# Autodesk Inventor assembly: Assembly2 (Intake Pipe Sub Assembly)
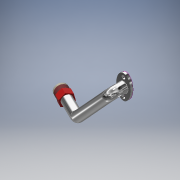
[picture p0: Inventor's stored thumbnail of the model, 180x180]
Saved by Autodesk Inventor 2018 (Build 220112000, 112)
## iProperties
Created: 2023-04-15
Part Number: Assembly2 (Intake Pipe Sub Assembly)
Document SubType Name: Assembly
Designer: Habib Mohamed
Author: Habib Mohamed
## Documents named in this file (5)
- D:\Inventor\My projects\Rotary Engine\Assembly\Assembly2 (Intake Pipe Sub Assembly).iam
- D:\Inventor\My projects\Rotary Engine\Component 51(Intake Pipe).ipt
- D:\Inventor\My projects\Rotary Engine\Component 29 (Flange Seal).ipt
- D:\Inventor\My projects\Rotary Engine\Component 30(Intake Pipe Ring).ipt
- D:\Inventor\My projects\Rotary Engine\Component 33(Intake Pipe Union).ipt
## Components (4 placed, 4 different names)
1. Component 51(Intake Pipe):1 — Mate:1, Mate:2, Mate:3, Mate:4, Mate:5, Flush:1
2. Component 29 (Flange Seal):1 — Mate:1, Mate:2, Mate:3
3. Component 30(Intake Pipe Ring):1 — Mate:5, Mate:6, Flush:1
4. Component 33(Intake Pipe Union):1 — Mate:4, Mate:6
## Relationships (7: Mate 6, Flush 1)
- Mate:1: Component 51(Intake Pipe):1 ↔ Component 29 (Flange Seal):1
- Mate:2: Component 51(Intake Pipe):1 ↔ Component 29 (Flange Seal):1
- Mate:3: Component 51(Intake Pipe):1 ↔ Component 29 (Flange Seal):1
- Mate:4: Component 51(Intake Pipe):1 ↔ Component 33(Intake Pipe Union):1
- Mate:5: Component 51(Intake Pipe):1 ↔ Component 30(Intake Pipe Ring):1
- Mate:6: Component 30(Intake Pipe Ring):1 ↔ Component 33(Intake Pipe Union):1
- Flush:1: Component 51(Intake Pipe):1 ↔ Component 30(Intake Pipe Ring):1
